# Autodesk Inventor assembly: Z Rail Right
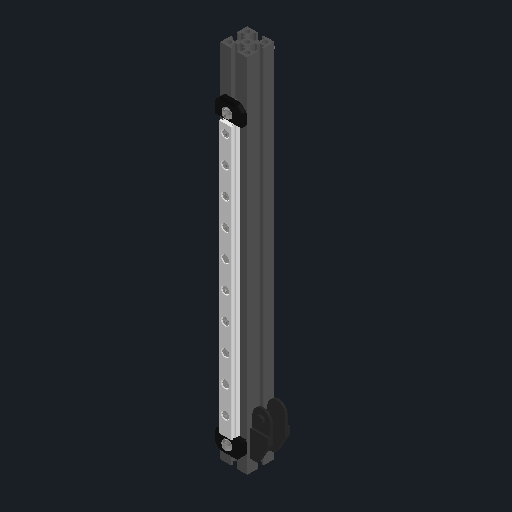
[picture p0: Inventor's stored thumbnail of the model, 512x512]
Saved by Autodesk Inventor 2025.1 (Build 291241020, 241B)
## iProperties
Created: 2025-05-11
Part Number: Z Rail Right
Document SubType Name: Assembly
Designer: Joshua Eah
Author: Joshua Eah
## Documents named in this file (9)
- C:\Users\Joshua Eah\Documents\Voron 0.2\CAD\Master Assembly\Frame\Subassemblies\Z Extrusion Right.iam
- Z Extrusion Right.iam
- C:\Users\Joshua Eah\Documents\Voron 0.2\CAD\Master Assembly\Frame\Parts\Extrusions\1515_200mm - C.ipt
- C:\Users\Joshua Eah\Documents\Voron 0.2\CAD\Master Assembly\Hardware\M3x6 BHCS.ipt
- C:\Users\Joshua Eah\Documents\Voron 0.2\CAD\Master Assembly\Hardware\M3 Hexnut.ipt
- C:\Users\Joshua Eah\Documents\Voron 0.2\CAD\Master Assembly\Linear Rail\MGN7 Rail 150mm.iam
- MGN7 150mm Rail.iam
- C:\Users\Joshua Eah\Documents\Voron 0.2\CAD\Master Assembly\Frame\Subassemblies\Rail Stop.iam
- C:\Users\Joshua Eah\Documents\Voron 0.2\CAD\Master Assembly\Chain Link End.iam
## Components (9 placed, 6 different names)
1. 1515_200mm - C:4
2. MGN7 Rail 150mm:2 [sub-assembly]
3. Rail Stop:2 [sub-assembly]
4. Rail Stop:3 [sub-assembly]
5. Chain Link End:1 [sub-assembly]
6. M3x6 BHCS:1
7. M3 Hexnut:8
8. M3 Hexnut:5
9. M3x6 BHCS:2
## Relationships (17: Mate 11, Flush 4, Insert 2)
- [Mate]: 1515_200mm - C:4 ↔ M3x6 BHCS:1
- [Mate]: 1515_200mm - C:4 ↔ M3x6 BHCS:1
- [Insert]: M3x6 BHCS:1 ↔ M3 Hexnut:8
- [Mate]: 1515_200mm - C:4 ↔ M3x6 BHCS:2
- [Mate]: 1515_200mm - C:4 ↔ M3x6 BHCS:2
- [Insert]: M3 Hexnut:5 ↔ M3x6 BHCS:2
- [Mate]: 1515_200mm - C:4 ↔ MGN7 Rail 150mm:2
- [Flush] (33 mm): 1515_200mm - C:4 ↔ MGN7 Rail 150mm:2
- [Mate] (0.1 mm): 1515_200mm - C:4 ↔ MGN7 Rail 150mm:2
- [Mate]: 1515_200mm - C:4 ↔ Rail Stop:2
- [Mate]: MGN7 Rail 150mm:2 ↔ Rail Stop:2
- [Flush]: 1515_200mm - C:4 ↔ Rail Stop:2
- [Mate]: MGN7 Rail 150mm:2 ↔ Rail Stop:3
- [Mate]: 1515_200mm - C:4 ↔ Rail Stop:3
- [Flush]: 1515_200mm - C:4 ↔ Rail Stop:3
- [Flush]: Rail Stop:3 ↔ Chain Link End:1
- [Mate]: 1515_200mm - C:4 ↔ Chain Link End:1
## Named parameters: d9_d12 = 33 mm, d14_d19 = 0 mm, d16_d20 = 0 mm
